# Autodesk Inventor assembly: 雙組合窗_MIR1
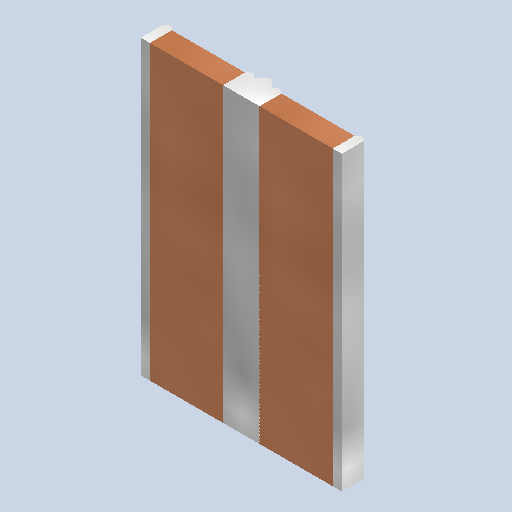
[picture p0: Inventor's stored thumbnail of the model, 512x512]
Saved by Autodesk Inventor 2024.2 (Build 282272000, 272)
## iProperties
Created: 2024-06-02
Part Number: 雙組合窗_MIR1
Document SubType Name: Assembly
Designer: User
Author: User
## Documents named in this file (4)
- C:\Users\User\OneDrive - 國立中山大學\桌面\創客基礎\final_project\mirror\雙組合窗_MIR1.iam
- C:\Users\User\OneDrive - 國立中山大學\桌面\創客基礎\final_project\mirror\窗_MIR1.ipt
- C:\Users\User\OneDrive - 國立中山大學\桌面\創客基礎\final_project\mirror\窗側柱_MIR1.ipt
- C:\Users\User\OneDrive - 國立中山大學\桌面\創客基礎\final_project\mirror\窗間柱_MIR1.ipt
## Components (5 placed, 3 different names)
1. 窗_MIR1:1 — 齊平:8, 齊平:7, 貼合:4, 齊平:2, 齊平:1, 貼合:2
2. 窗_MIR1:2 — 齊平:6, 齊平:5, 貼合:3, 齊平:4, 齊平:3, 貼合:1
3. 窗側柱_MIR1:1 — 齊平:8, 齊平:7, 貼合:4
4. 窗側柱_MIR1:2 — 齊平:6, 齊平:5, 貼合:3
5. 窗間柱_MIR1:1 — 齊平:4, 齊平:3, 齊平:2, 齊平:1, 貼合:2, 貼合:1
## Relationships (12: Flush 8, Mate 4)
- 齊平:8 [Flush]: 窗_MIR1:1 ↔ 窗側柱_MIR1:1
- 齊平:7 [Flush]: 窗_MIR1:1 ↔ 窗側柱_MIR1:1
- 貼合:4 [Mate]: 窗_MIR1:1 ↔ 窗側柱_MIR1:1
- 齊平:6 [Flush]: 窗_MIR1:2 ↔ 窗側柱_MIR1:2
- 齊平:5 [Flush]: 窗_MIR1:2 ↔ 窗側柱_MIR1:2
- 貼合:3 [Mate]: 窗_MIR1:2 ↔ 窗側柱_MIR1:2
- 齊平:4 [Flush]: 窗_MIR1:2 ↔ 窗間柱_MIR1:1
- 齊平:3 [Flush]: 窗_MIR1:2 ↔ 窗間柱_MIR1:1
- 齊平:2 [Flush]: 窗_MIR1:1 ↔ 窗間柱_MIR1:1
- 齊平:1 [Flush]: 窗_MIR1:1 ↔ 窗間柱_MIR1:1
- 貼合:2 [Mate]: 窗_MIR1:1 ↔ 窗間柱_MIR1:1
- 貼合:1 [Mate]: 窗_MIR1:2 ↔ 窗間柱_MIR1:1
